# Autodesk Inventor assembly: CO-0-01-controlsBox
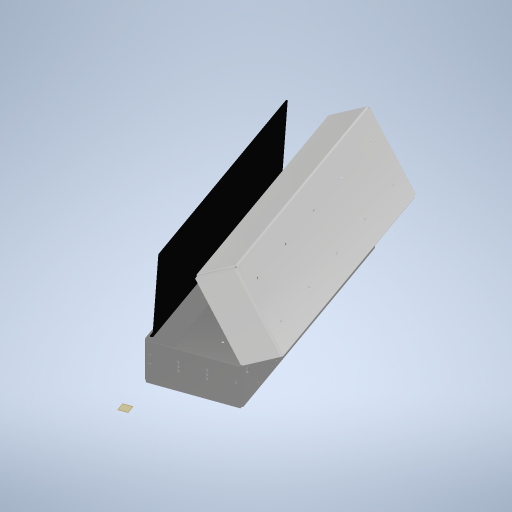
[picture p0: Inventor's stored thumbnail of the model, 512x512]
Saved by Autodesk Inventor 2023 (Build 270158000, 158)
## iProperties
Created: 2023-04-11
Part Number: CO-0-01-controlsBox
Document SubType Name: Weldment
Designer: t205b
Weld Material: Welded Aluminum-6061
Author: t205b
## Documents named in this file (4)
- C:\Users\t205b\OneDrive\Documents\PSU Extracuriculars\Robotics\URC Electrical\CO-0-01-controlsBox.iam
- C:\Users\t205b\OneDrive\Documents\PSU Extracuriculars\Robotics\URC Electrical\CO-1-02-controlsBox.ipt
- C:\Users\t205b\OneDrive\Documents\PSU Extracuriculars\Robotics\URC Electrical\CO-1-01-controlsSeperator.ipt
- C:\Users\t205b\OneDrive\Documents\PSU Extracuriculars\Robotics\URC Electrical\CO-1-01-controlsLid.ipt
## Components (3 placed, 3 different names)
1. CO-1-02-controlsBox:1 — Cylindrical:1, Flush:1, Cylindrical:2, Mate:1, Mate:2
2. CO-1-01-controlsSeperator:1 — Cylindrical:2, Mate:1
3. CO-1-01-controlsLid:1 — Cylindrical:1, Flush:1
## Relationships (5: CylindricalJoint 2, Mate 2, Flush 1)
- Cylindrical:1: CO-1-02-controlsBox:1 ↔ CO-1-01-controlsLid:1
- Flush:1: CO-1-02-controlsBox:1 ↔ CO-1-01-controlsLid:1
- Cylindrical:2: CO-1-02-controlsBox:1 ↔ CO-1-01-controlsSeperator:1
- Mate:1: CO-1-02-controlsBox:1 ↔ CO-1-01-controlsSeperator:1
- Mate:2: CO-1-02-controlsBox:1
